# Autodesk Inventor assembly: clapper box assembly
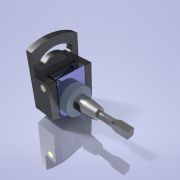
[picture p0: Inventor's stored thumbnail of the model, 180x180]
Saved by Autodesk Inventor 2021.1 (Build 251245000, 245)
## iProperties
Created: 2021-02-18
Part Number: clapper box assembly
Document SubType Name: Assembly
Designer: Vamshi
Author: Vamshi
## Documents named in this file (7)
- B:\project\clapper box\clapper box assembly.iam
- B:\project\clapper box\swivel plate.ipt
- B:\project\clapper box\drag release plate.ipt
- B:\project\clapper box\pin.ipt
- B:\project\clapper box\tool holder.ipt
- B:\project\clapper box\washer.ipt
- B:\project\clapper box\tool clamping screw.ipt
## Components (6 placed, 6 different names)
1. swivel plate:1 — Mate:1, Mate:2, Mate:3, Mate:4
2. drag release plate:1 — Mate:1, Mate:2, Mate:5, Mate:6, Mate:8
3. pin:1 — Mate:3, Mate:4
4. tool holder:1 — Mate:5, Mate:6, Mate:7, Mate:9
5. washer:1 — Mate:7, Mate:8
6. tool clamping screw:1 — Mate:9
## Relationships (9: Mate 9)
- Mate:1: swivel plate:1 ↔ drag release plate:1
- Mate:2: swivel plate:1 ↔ drag release plate:1
- Mate:3: swivel plate:1 ↔ pin:1
- Mate:4: swivel plate:1 ↔ pin:1
- Mate:5: drag release plate:1 ↔ tool holder:1
- Mate:6: drag release plate:1 ↔ tool holder:1
- Mate:7: tool holder:1 ↔ washer:1
- Mate:8: drag release plate:1 ↔ washer:1
- Mate:9: tool holder:1 ↔ tool clamping screw:1
